# Autodesk Inventor assembly: RailAttachmentAssemblyLeftWithoutPi
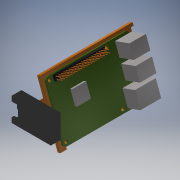
[picture p0: Inventor's stored thumbnail of the model, 180x180]
Saved by Autodesk Inventor 2018 (Build 220112000, 112)
## iProperties
Created: 2019-04-01
Part Number: RailAttachmentAssemblyLeftWithoutPi
Document SubType Name: Assembly
Designer: snipe
Author: snipe
## Documents named in this file (4)
- C:\Users\snipe\Documents\CPRE186-CAD\RailAttachmentAssemblyLeft.iam
- C:\Users\snipe\Documents\CPRE186-CAD\nerfRailMount.ipt
- C:\Users\snipe\Documents\CPRE186-CAD\Raspi3B+_Case.ipt
- C:\Users\snipe\Documents\CPRE186-CAD\Raspi3B+_Mockup.ipt
## Components (3 placed, 3 different names)
1. nerfRailMount:1 — Angle:1, Mate:7, Mate:8, Mate:9
2. Raspi3B+_Case:1 — Angle:1, Mate:7, Mate:8, Mate:9, Mate:10, Mate:11, Mate:12
3. Raspi3B+_Mockup:1 — Mate:10, Mate:11, Mate:12
## Relationships (7: Mate 6, Angle 1)
- Angle:1 (290 deg): nerfRailMount:1 ↔ Raspi3B+_Case:1
- Mate:7: nerfRailMount:1 ↔ Raspi3B+_Case:1
- Mate:8: nerfRailMount:1 ↔ Raspi3B+_Case:1
- Mate:9 (12.7 mm): nerfRailMount:1 ↔ Raspi3B+_Case:1
- Mate:10: Raspi3B+_Case:1 ↔ Raspi3B+_Mockup:1
- Mate:11: Raspi3B+_Case:1 ↔ Raspi3B+_Mockup:1
- Mate:12: Raspi3B+_Case:1 ↔ Raspi3B+_Mockup:1
